# Autodesk Inventor assembly: Battery Holder Assembly
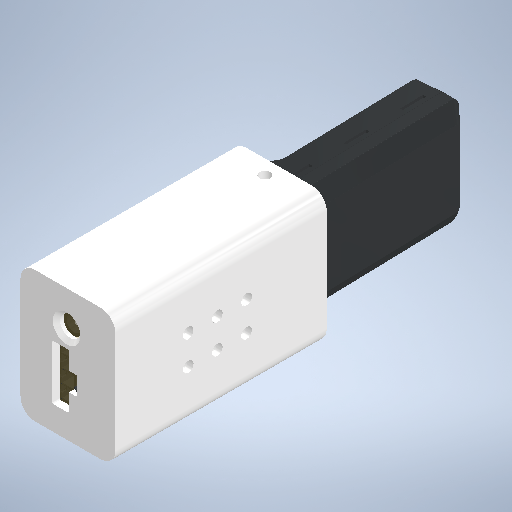
[picture p0: Inventor's stored thumbnail of the model, 512x512]
Saved by Autodesk Inventor 2025.1 (Build 291241020, 241B)
## iProperties
Created: 2024-12-04
Part Number: Battery Holder Assembly
Document SubType Name: Assembly
Designer: AtuStem
Author: AtuStem
## Documents named in this file (3)
- C:\Users\AtuStem\Documents\GitHub\ATUM-V5RC-High-Stakes-CAD\Battery Holder Assembly.iam
- C:\Users\AtuStem\Documents\GitHub\ATUM-V5RC-High-Stakes-CAD\VEX-CAD-Inventor\Electronics\V5 Battery.ipt
- C:\Users\AtuStem\Documents\GitHub\ATUM-V5RC-High-Stakes-CAD\Additional Parts\Battery Holder.ipt
## Components (2 placed, 2 different names)
1. V5 Battery:1 — Rigid:1
2. Battery Holder:1 — Rigid:1
## Relationships (1: WeldJoint 1)
- Rigid:1 [WeldJoint]: V5 Battery:1 ↔ Battery Holder:1
